# Autodesk Inventor assembly: Chalk Applicator
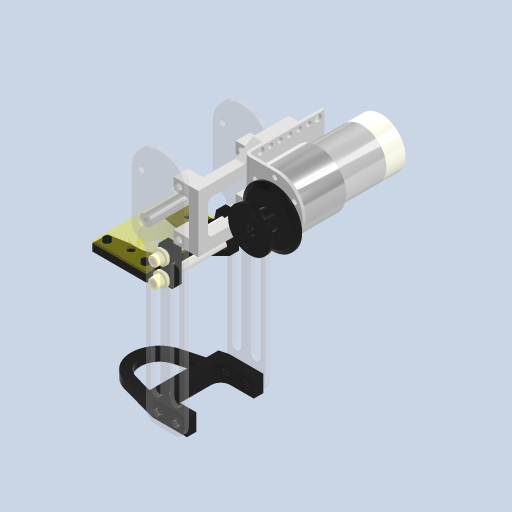
[picture p0: Inventor's stored thumbnail of the model, 512x512]
Saved by Autodesk Inventor 2024 (Build 280153000, 153)
## iProperties
Created: 2023-12-18
Part Number: Chalk Applicator
Document SubType Name: Assembly
Designer: greg
Author: greg
## Documents named in this file (14)
- C:\Users\Greg\Documents\Inventor\Capstone\Chalk Applicator\Chalk Applicator.iam
- C:\Users\Greg\Documents\Inventor\Capstone\Chalk Applicator\Cross Shaft.iam
- C:\Users\Greg\Documents\Inventor\Capstone\Chalk Applicator\Side Plate.ipt
- C:\Users\Greg\Documents\Inventor\Capstone\Chalk Applicator\Standoff.ipt
- C:\Users\greg\Documents\Inventor\Content Center Files\R2024\en-US\ANSI B18.6.3(60)\ANSI B18.6.3 - 6-32 UNC - 1.25(25).ipt
- C:\Users\Greg\Documents\Inventor\Capstone\Chalk Applicator\Vince-Motor.iam
- C:\Users\Greg\Documents\Inventor\Capstone\Chalk Applicator\Pulley.ipt
- C:\Users\Greg\Documents\Inventor\Capstone\Chalk Applicator\Carriage.ipt
- C:\Users\Greg\Documents\Inventor\Capstone\Chalk Applicator\Gripper.ipt
- C:\Users\greg\Documents\Inventor\Content Center Files\R2024\en-US\ANSI B18.6.3(24)\ANSI B18.6.3 - 10-24 UNC - 0.4375(4A).ipt
- C:\Users\greg\Documents\Inventor\Content Center Files\R2024\en-US\ANSI B18.22.1\ANSI B18.22.1 - No. 10 - Type A.ipt
- C:\Users\greg\Documents\Inventor\Content Center Files\R2024\en-US\ANSI B18.17(12)\ANSI B18.17 - No. 10 - 24 Light SeriesA (1).ipt
- C:\Users\Greg\Documents\Inventor\Capstone\Chalk Applicator\Lower Guide.ipt
- C:\Users\Greg\Documents\Inventor\Capstone\Chalk Applicator\Rear Plate.ipt
## Components (27 placed, 13 different names)
1. Side Plate:1 — Insert:8, Mate:21, Tangent:1, Mate:22, Tangent:2, Mate:39, Mate:40, Mate:41, Mate:42, Mate:43, Mate:44, Mate:45, Mate:46, Mate:47, Mate:48, Insert:19, Insert:20
2. Side Plate:2 — Insert:4, Mate:11, Mate:12, Mate:13, Mate:14, Mate:15, Mate:16, Mate:17, Mate:18, Mate:19, Mate:20, Mate:23, Mate:24, Flush:1, Mate:49, Mate:50, Insert:17, Insert:18
3. Cross Shaft:1 [sub-assembly] — Mate:22, Tangent:2, Mate:23, Mate:29
4. Cross Shaft:2 [sub-assembly] — Mate:21, Tangent:1, Mate:24, Mate:28, Mate:30
5. Standoff:4 — Insert:4, Insert:8
6. Square Recessed Pan Head Machine Screw - Type III - Inch (IFI) 6-32 UNC - 1.25:1 — Mate:39, Mate:40
7. Square Recessed Pan Head Machine Screw - Type III - Inch (IFI) 6-32 UNC - 1.25:6 — Mate:11, Mate:12
8. Square Recessed Pan Head Machine Screw - Type III - Inch (IFI) 6-32 UNC - 1.25:7 — Mate:13, Mate:14
9. Square Recessed Pan Head Machine Screw - Type III - Inch (IFI) 6-32 UNC - 1.25:8 — Mate:15, Mate:16
10. Square Recessed Pan Head Machine Screw - Type III - Inch (IFI) 6-32 UNC - 1.25:9 — Mate:17, Mate:18
11. Square Recessed Pan Head Machine Screw - Type III - Inch (IFI) 6-32 UNC - 1.25:10 — Mate:19, Mate:20
12. Carriage:1 — Mate:28, Mate:29, Mate:30, Insert:11, Insert:12, Mate:31, Mate:32, Mate:33, Mate:34, Mate:35, Mate:37
13. Gripper:1 — Insert:11, Insert:12, Mate:36, Mate:38
14. Lower Guide:1 — Flush:1
15. Cross Recessed Pan Head Machine Screw - Type I - Inch No. 10 - 24 - 7/16:1 — Mate:31, Mate:32
16. Plain Washer (Inch) No. 10 - Type A:1 — Mate:35, Mate:36, Insert:13
17. Type A - Wing Nut - Inch No. 10 - 24 Light Series:1 — Insert:13
18. Cross Recessed Pan Head Machine Screw - Type I - Inch No. 10 - 24 - 7/16:2 — Mate:33, Mate:34
19. Plain Washer (Inch) No. 10 - Type A:2 — Mate:37, Mate:38, Insert:14
20. Type A - Wing Nut - Inch No. 10 - 24 Light Series:2 — Insert:14
21. Square Recessed Pan Head Machine Screw - Type III - Inch (IFI) 6-32 UNC - 1.25:11 — Mate:41, Mate:42
22. Square Recessed Pan Head Machine Screw - Type III - Inch (IFI) 6-32 UNC - 1.25:12 — Mate:43, Mate:44
23. Square Recessed Pan Head Machine Screw - Type III - Inch (IFI) 6-32 UNC - 1.25:13 — Mate:45, Mate:46
24. Square Recessed Pan Head Machine Screw - Type III - Inch (IFI) 6-32 UNC - 1.25:14 — Mate:47, Mate:48
25. Pulley:1 — Insert:21
26. Vince-Motor:1 [sub-assembly] — Insert:15, Insert:16, Insert:21
27. Rear Plate:1 — Insert:15, Insert:16, Mate:49, Mate:50, Insert:17, Insert:18, Insert:19, Insert:20
## Relationships (53: Mate 37, Insert 13, Tangent 2, Flush 1)
- Insert:4: Side Plate:2 ↔ Standoff:4
- Insert:8: Side Plate:1 ↔ Standoff:4
- Mate:11: Side Plate:2 ↔ Square Recessed Pan Head Machine Screw - Type III - Inch (IFI) 6-32 UNC - 1.25:6
- Mate:12: Side Plate:2 ↔ Square Recessed Pan Head Machine Screw - Type III - Inch (IFI) 6-32 UNC - 1.25:6
- Mate:13: Side Plate:2 ↔ Square Recessed Pan Head Machine Screw - Type III - Inch (IFI) 6-32 UNC - 1.25:7
- Mate:14: Side Plate:2 ↔ Square Recessed Pan Head Machine Screw - Type III - Inch (IFI) 6-32 UNC - 1.25:7
- Mate:15: Side Plate:2 ↔ Square Recessed Pan Head Machine Screw - Type III - Inch (IFI) 6-32 UNC - 1.25:8
- Mate:16: Side Plate:2 ↔ Square Recessed Pan Head Machine Screw - Type III - Inch (IFI) 6-32 UNC - 1.25:8
- Mate:17: Side Plate:2 ↔ Square Recessed Pan Head Machine Screw - Type III - Inch (IFI) 6-32 UNC - 1.25:9
- Mate:18: Side Plate:2 ↔ Square Recessed Pan Head Machine Screw - Type III - Inch (IFI) 6-32 UNC - 1.25:9
- Mate:19: Side Plate:2 ↔ Square Recessed Pan Head Machine Screw - Type III - Inch (IFI) 6-32 UNC - 1.25:10
- Mate:20: Side Plate:2 ↔ Square Recessed Pan Head Machine Screw - Type III - Inch (IFI) 6-32 UNC - 1.25:10
- Mate:21: Side Plate:1 ↔ Cross Shaft:2
- Tangent:1: Side Plate:1 ↔ Cross Shaft:2
- Mate:22: Side Plate:1 ↔ Cross Shaft:1
- Tangent:2: Side Plate:1 ↔ Cross Shaft:1
- Mate:23: Side Plate:2 ↔ Cross Shaft:1
- Mate:24: Side Plate:2 ↔ Cross Shaft:2
- Mate:28: Cross Shaft:2 ↔ Carriage:1
- Mate:29: Cross Shaft:1 ↔ Carriage:1
- Mate:30 (1.5875 mm): Cross Shaft:2 ↔ Carriage:1
- Insert:11: Carriage:1 ↔ Gripper:1
- Insert:12: Carriage:1 ↔ Gripper:1
- Mate:31: Carriage:1 ↔ Cross Recessed Pan Head Machine Screw - Type I - Inch No. 10 - 24 - 7/16:1
- Mate:32: Carriage:1 ↔ Cross Recessed Pan Head Machine Screw - Type I - Inch No. 10 - 24 - 7/16:1
- Mate:33: Carriage:1 ↔ Cross Recessed Pan Head Machine Screw - Type I - Inch No. 10 - 24 - 7/16:2
- Mate:34: Carriage:1 ↔ Cross Recessed Pan Head Machine Screw - Type I - Inch No. 10 - 24 - 7/16:2
- Mate:35: Carriage:1 ↔ Plain Washer (Inch) No. 10 - Type A:1
- Mate:36: Gripper:1 ↔ Plain Washer (Inch) No. 10 - Type A:1
- Mate:37: Carriage:1 ↔ Plain Washer (Inch) No. 10 - Type A:2
- Mate:38: Gripper:1 ↔ Plain Washer (Inch) No. 10 - Type A:2
- Insert:13: Plain Washer (Inch) No. 10 - Type A:1 ↔ Type A - Wing Nut - Inch No. 10 - 24 Light Series:1
- Insert:14: Plain Washer (Inch) No. 10 - Type A:2 ↔ Type A - Wing Nut - Inch No. 10 - 24 Light Series:2
- Flush:1: Side Plate:2 ↔ Lower Guide:1
- Mate:39: Side Plate:1 ↔ Square Recessed Pan Head Machine Screw - Type III - Inch (IFI) 6-32 UNC - 1.25:1
- Mate:40: Side Plate:1 ↔ Square Recessed Pan Head Machine Screw - Type III - Inch (IFI) 6-32 UNC - 1.25:1
- Mate:41: Side Plate:1 ↔ Square Recessed Pan Head Machine Screw - Type III - Inch (IFI) 6-32 UNC - 1.25:11
- Mate:42: Side Plate:1 ↔ Square Recessed Pan Head Machine Screw - Type III - Inch (IFI) 6-32 UNC - 1.25:11
- Mate:43: Side Plate:1 ↔ Square Recessed Pan Head Machine Screw - Type III - Inch (IFI) 6-32 UNC - 1.25:12
- Mate:44: Side Plate:1 ↔ Square Recessed Pan Head Machine Screw - Type III - Inch (IFI) 6-32 UNC - 1.25:12
- Mate:45: Side Plate:1 ↔ Square Recessed Pan Head Machine Screw - Type III - Inch (IFI) 6-32 UNC - 1.25:13
- Mate:46: Side Plate:1 ↔ Square Recessed Pan Head Machine Screw - Type III - Inch (IFI) 6-32 UNC - 1.25:13
- Mate:47: Side Plate:1 ↔ Square Recessed Pan Head Machine Screw - Type III - Inch (IFI) 6-32 UNC - 1.25:14
- Mate:48: Side Plate:1 ↔ Square Recessed Pan Head Machine Screw - Type III - Inch (IFI) 6-32 UNC - 1.25:14
- Insert:15: Vince-Motor:1 ↔ Rear Plate:1
- Insert:16: Vince-Motor:1 ↔ Rear Plate:1
- Mate:49: Side Plate:2 ↔ Rear Plate:1
- Mate:50: Side Plate:2 ↔ Rear Plate:1
- Insert:17: Side Plate:2 ↔ Rear Plate:1
- Insert:18: Side Plate:2 ↔ Rear Plate:1
- Insert:19: Side Plate:1 ↔ Rear Plate:1
- Insert:20: Side Plate:1 ↔ Rear Plate:1
- Insert:21: Pulley:1 ↔ Vince-Motor:1
